# Autodesk Inventor assembly: Celdas
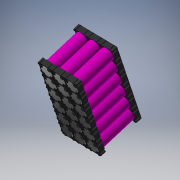
[picture p0: Inventor's stored thumbnail of the model, 180x180]
Saved by Autodesk Inventor 2018.3 (Build 223285000, 285)
## iProperties
Created: 2020-11-27
Part Number: Celdas
Material: Genérico
Document SubType Name: Assembly
Designer: felip
Author: felip
## Documents named in this file (3)
- C:\Users\felip\Desktop\Taller\Celdas.iam
- C:\Users\felip\Desktop\Taller\Base_18650.ipt
- C:\Users\felip\Desktop\Taller\Pila_18650.ipt
## Components (54 placed, 2 different names)
1. Base_18650:3 — Insertar:1, Nivelación:1, Nivelación:2
2. Base_18650:4
3. Base_18650:5
4. Base_18650:6
5. Base_18650:7
6. Base_18650:8
7. Base_18650:9
8. Base_18650:10
9. Base_18650:11
10. Base_18650:12
11. Base_18650:13
12. Base_18650:14
13. Base_18650:15
14. Base_18650:16
15. Base_18650:17
16. Base_18650:18
17. Base_18650:19
18. Base_18650:20
19. Pila_18650:1 — Insertar:1, Coincidencia:1, Coincidencia:2
20. Pila_18650:2
21. Pila_18650:3
22. Pila_18650:4
23. Pila_18650:5
24. Pila_18650:6
25. Pila_18650:7
26. Pila_18650:8
27. Pila_18650:9
28. Pila_18650:10
29. Pila_18650:11
30. Pila_18650:12
31. Pila_18650:13
32. Pila_18650:14
33. Pila_18650:15
34. Pila_18650:16
35. Pila_18650:17
36. Pila_18650:18
37. Base_18650:21 — Coincidencia:1, Nivelación:1, Coincidencia:2, Nivelación:2
38. Base_18650:22
39. Base_18650:23
40. Base_18650:24
41. Base_18650:25
42. Base_18650:26
43. Base_18650:27
44. Base_18650:28
45. Base_18650:29
46. Base_18650:30
47. Base_18650:31
48. Base_18650:32
49. Base_18650:33
50. Base_18650:34
51. Base_18650:35
52. Base_18650:36
53. Base_18650:37
54. Base_18650:38
## Component patterns: (18 elements, first: Base_18650:3), (18 elements, first: Pila_18650:1), (18 elements, first: Base_18650:21)
## Relationships (5: Mate 2, Flush 2, Insert 1)
- Insertar:1: Base_18650:3 ↔ Pila_18650:1
- Coincidencia:1 [Mate]: Pila_18650:1 ↔ Base_18650:21
- Nivelación:1 [Flush]: Base_18650:3 ↔ Base_18650:21
- Coincidencia:2 [Mate]: Pila_18650:1 ↔ Base_18650:21
- Nivelación:2 [Flush]: Base_18650:3 ↔ Base_18650:21
